# Autodesk Inventor assembly: KeySwitch
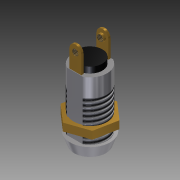
[picture p0: Inventor's stored thumbnail of the model, 180x180]
Saved by Autodesk Inventor 2015 SP1 (Build 190203100, 203)
## iProperties
Created: 2015-01-26
Part Number: KeySwitch
Document SubType Name: Assembly
Designer: Jack
Mass: 83.898 g
Surface Area: 47.172 cm^2
Volume: 11.4558 cm^3
Density: 7.32365 g/cm^3
Author: Jack
Title: Key Switch
## Documents named in this file (3)
- C:\Users\Jack\ownCloud\Projects\CrossBot\InventorModel\Electronics\KeySwitch\KeySwitch.iam
- C:\Users\Jack\ownCloud\Projects\CrossBot\InventorModel\Electronics\KeySwitch\KeySwitchBody.ipt
- C:\Users\Jack\ownCloud\Projects\CrossBot\InventorModel\Electronics\KeySwitch\KeySwitchNut.ipt
## Components (2 placed, 2 different names)
1. KeySwitchBody:1 — Mate:1, Mate:2
2. KeySwitchNut:1 — Mate:1, Mate:2
## Relationships (2: Mate 2)
- Mate:1: KeySwitchBody:1 ↔ KeySwitchNut:1
- Mate:2 (4.7625 mm): KeySwitchBody:1 ↔ KeySwitchNut:1
